# Autodesk Inventor assembly: Wind Tunnel Inlet Test Assembly (To Simulate)
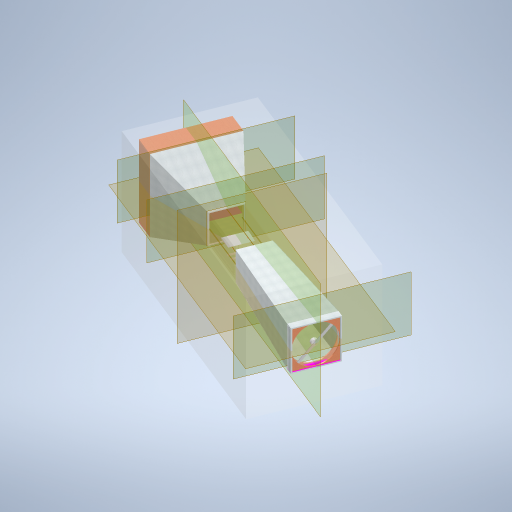
[picture p0: Inventor's stored thumbnail of the model, 512x512]
Saved by Autodesk Inventor 2023 (Build 270158000, 158)
## iProperties
Created: 2022-01-10
Part Number: Wind Tunnel Inlet Test Assembly (To Simulate)
Document SubType Name: Assembly
Designer: kamer
Author: kamer
## iProperties of the stored document MemberDocs/xAaaaqwbaAaaaaaaaAaaaavk0Cc
Created: 2022-01-10
Part Number: Wind Tunnel Inlet Test Assembly (To Simulate)
Document SubType Name: Assembly
Designer: kamer
Author: kamer
## Documents named in this file (21)
- X:\Storage\Documents\ME 306 Heat Transfer Project Files\CAD\Main With Subparts.iam
- X:\Storage\Documents\ME 306 Heat Transfer Project Files\CAD\Wind Tunnel Inlet Body Single Panel.ipt
- X:\Storage\Documents\ME 306 Heat Transfer Project Files\CAD\Wind Tunnel Output Body Single Panel.ipt
- X:\Storage\Documents\ME 306 Heat Transfer Project Files\CAD\Test Section Assembly.iam
- X:\Storage\Documents\ME 306 Heat Transfer Project Files\CAD\Fluid Simulation Boundary.ipt
- X:\Storage\Documents\ME 306 Heat Transfer Project Files\CAD\Wind Tunnel Settling Chamber.iam
- X:\Storage\Documents\ME 306 Heat Transfer Project Files\CAD\Wind Tunnel Exhaust Frame.iam
- X:\Storage\Documents\ME 306 Heat Transfer Project Files\CAD\Motor Mockup.ipt
- X:\Storage\Documents\ME 306 Heat Transfer Project Files\CAD\Wind Tunnel Fan Shroud Corner.ipt
- X:\Storage\Documents\ME 306 Heat Transfer Project Files\CAD\Motor Strap.ipt
- X:\Storage\Documents\ME 306 Heat Transfer Project Files\CAD\Wind Tunnel Exhaust Frame As-built.iam
- X:\Storage\Documents\ME 306 Heat Transfer Project Files\CAD\Wind Tunnel Inlet Body Single Panel Graphic Only.ipt
- X:\Storage\Documents\ME 306 Heat Transfer Project Files\CAD\Wind Tunnel Output Body Single Panel Graphic Only.ipt
- X:\Storage\Documents\ME 306 Heat Transfer Project Files\CAD\Wind Tunnel Settling Chamber As-Built.iam
- X:\Storage\Documents\ME 306 Heat Transfer Project Files\CAD\Inlet Support Leg Proto 1.ipt
- X:\Storage\Documents\ME 306 Heat Transfer Project Files\CAD\Outlet Support Leg Proto 1.ipt
- X:\Storage\Documents\ME 306 Heat Transfer Project Files\CAD\Computer Box Assembly Rev2.iam
- X:\Storage\Documents\ME 306 Heat Transfer Project Files\CAD\PowerBoardAssembly.iam
- X:\Storage\Documents\ME 306 Heat Transfer Project Files\CAD\Antitorque Outlet Support.ipt
- X:\Storage\Documents\ME 306 Heat Transfer Project Files\CAD\Antitorque span.ipt
- X:\Storage\Documents\ME 306 Heat Transfer Project Files\CAD\Antitorque leg-leg span.ipt
## Components (22 placed, 9 different names)
1. Wind Tunnel Inlet Body Single Panel:1 — Mate:1, Mate:3, Angle:1, Mate:24
2. Wind Tunnel Inlet Body Single Panel:2 — Mate:1, Mate:2, Angle:1, Mate:22, Mate:30, Mate:33
3. Wind Tunnel Inlet Body Single Panel:3 — Mate:2, Mate:4, Mate:14, Mate:23, Mate:32
4. Wind Tunnel Inlet Body Single Panel:4 — Mate:3, Mate:4, Mate:13, Mate:15, Mate:27
5. Wind Tunnel Output Body Single Panel:1 — Mate:16, Mate:17, Mate:22, Mate:35
6. Wind Tunnel Output Body Single Panel:2 — Mate:18, Mate:19, Mate:24, Mate:34
7. Wind Tunnel Output Body Single Panel:3 — Mate:25, Mate:26, Mate:27
8. Wind Tunnel Output Body Single Panel:4 — Mate:20, Mate:21, Mate:23
9. Test Section Assembly:1 [sub-assembly] — Mate:13, Mate:14, Mate:15, Mate:16, Mate:17, Mate:18, Mate:19, Mate:20, Mate:21, Mate:25, Mate:26, Mate:28, Mate:29, Angle:2
10. Fluid Simulation Boundary:1 — Mate:28, Mate:29
11. Wind Tunnel Settling Chamber:1 [sub-assembly] — Mate:31, Mate:32, Mate:33
12. Wind Tunnel Exhaust Frame:1 [sub-assembly] — Flush:3, Mate:34, Mate:35, Mate:36, Mate:37, Flush:4, Mate:38, Mate:39, Mate:40, Mate:41, Mate:42, Mate:43, Mate:47, Mate:48, Mate:50, Mate:51, Mate:52, Mate:53, Mate:56, Mate:57, Mate:58, Mate:59
13. Motor Mockup:1 — Mate:44, Mate:45, Mate:49
14. Wind Tunnel Fan Shroud Corner:1 — Mate:36, Mate:37, Flush:4, Flush:5, Mate:45
15. Wind Tunnel Fan Shroud Corner:2 — Mate:42, Mate:43, Flush:7, Mate:44
16. Wind Tunnel Fan Shroud Corner:3 — Mate:40, Mate:41, Flush:6, Flush:7
17. Wind Tunnel Fan Shroud Corner:4 — Mate:38, Mate:39, Flush:5, Flush:6
18. Motor Strap:1 — Mate:47, Mate:48, Mate:49, Mate:54, Mate:55
19. Wind Tunnel Fan Shroud Corner:5 — Mate:50, Mate:51, Mate:54, Flush:8
20. Wind Tunnel Fan Shroud Corner:6 — Mate:52, Mate:53, Mate:55, Flush:9
21. Wind Tunnel Fan Shroud Corner:7 — Mate:56, Mate:57, Flush:8
22. Wind Tunnel Fan Shroud Corner:8 — Mate:58, Mate:59, Flush:9
## Relationships (61: Mate 50, Flush 9, Angle 2)
- Mate:1: Wind Tunnel Inlet Body Single Panel:1 ↔ Wind Tunnel Inlet Body Single Panel:2
- Mate:2: Wind Tunnel Inlet Body Single Panel:2 ↔ Wind Tunnel Inlet Body Single Panel:3
- Mate:3: Wind Tunnel Inlet Body Single Panel:1 ↔ Wind Tunnel Inlet Body Single Panel:4
- Mate:4: Wind Tunnel Inlet Body Single Panel:3 ↔ Wind Tunnel Inlet Body Single Panel:4
- Angle:1 (90 deg): Wind Tunnel Inlet Body Single Panel:1 ↔ Wind Tunnel Inlet Body Single Panel:2
- Mate:13: Wind Tunnel Inlet Body Single Panel:4 ↔ Test Section Assembly:1
- Mate:14: Wind Tunnel Inlet Body Single Panel:3 ↔ Test Section Assembly:1
- Mate:15: Wind Tunnel Inlet Body Single Panel:4 ↔ Test Section Assembly:1
- Mate:16: Wind Tunnel Output Body Single Panel:1 ↔ Test Section Assembly:1
- Mate:17: Wind Tunnel Output Body Single Panel:1 ↔ Test Section Assembly:1
- Mate:18: Wind Tunnel Output Body Single Panel:2 ↔ Test Section Assembly:1
- Mate:19: Wind Tunnel Output Body Single Panel:2 ↔ Test Section Assembly:1
- Mate:20: Wind Tunnel Output Body Single Panel:4 ↔ Test Section Assembly:1
- Mate:21: Wind Tunnel Output Body Single Panel:4 ↔ Test Section Assembly:1
- Mate:22: Wind Tunnel Inlet Body Single Panel:2 ↔ Wind Tunnel Output Body Single Panel:1
- Mate:23: Wind Tunnel Inlet Body Single Panel:3 ↔ Wind Tunnel Output Body Single Panel:4
- Mate:24: Wind Tunnel Inlet Body Single Panel:1 ↔ Wind Tunnel Output Body Single Panel:2
- Mate:25: Wind Tunnel Output Body Single Panel:3 ↔ Test Section Assembly:1
- Mate:26: Wind Tunnel Output Body Single Panel:3 ↔ Test Section Assembly:1
- Mate:27: Wind Tunnel Inlet Body Single Panel:4 ↔ Wind Tunnel Output Body Single Panel:3
- Mate:28: Test Section Assembly:1 ↔ Fluid Simulation Boundary:1
- Mate:29: Test Section Assembly:1 ↔ Fluid Simulation Boundary:1
- Mate:30: Wind Tunnel Inlet Body Single Panel:2
- Angle:2 (90 deg): Test Section Assembly:1
- Flush:1 (617.22 mm)
- Mate:31: Wind Tunnel Settling Chamber:1
- Mate:32: Wind Tunnel Inlet Body Single Panel:3 ↔ Wind Tunnel Settling Chamber:1
- Mate:33: Wind Tunnel Inlet Body Single Panel:2 ↔ Wind Tunnel Settling Chamber:1
- Flush:2 (-1801.0886 mm)
- Flush:3: Wind Tunnel Exhaust Frame:1
- Mate:34: Wind Tunnel Output Body Single Panel:2 ↔ Wind Tunnel Exhaust Frame:1
- Mate:35: Wind Tunnel Output Body Single Panel:1 ↔ Wind Tunnel Exhaust Frame:1
- Mate:36: Wind Tunnel Exhaust Frame:1 ↔ Wind Tunnel Fan Shroud Corner:1
- Mate:37: Wind Tunnel Exhaust Frame:1 ↔ Wind Tunnel Fan Shroud Corner:1
- Flush:4 (63.5 mm): Wind Tunnel Exhaust Frame:1 ↔ Wind Tunnel Fan Shroud Corner:1
- Mate:38: Wind Tunnel Exhaust Frame:1 ↔ Wind Tunnel Fan Shroud Corner:4
- Mate:39: Wind Tunnel Exhaust Frame:1 ↔ Wind Tunnel Fan Shroud Corner:4
- Flush:5: Wind Tunnel Fan Shroud Corner:1 ↔ Wind Tunnel Fan Shroud Corner:4
- Mate:40: Wind Tunnel Exhaust Frame:1 ↔ Wind Tunnel Fan Shroud Corner:3
- Mate:41: Wind Tunnel Exhaust Frame:1 ↔ Wind Tunnel Fan Shroud Corner:3
- Flush:6: Wind Tunnel Fan Shroud Corner:3 ↔ Wind Tunnel Fan Shroud Corner:4
- Mate:42: Wind Tunnel Exhaust Frame:1 ↔ Wind Tunnel Fan Shroud Corner:2
- Mate:43: Wind Tunnel Exhaust Frame:1 ↔ Wind Tunnel Fan Shroud Corner:2
- Flush:7: Wind Tunnel Fan Shroud Corner:2 ↔ Wind Tunnel Fan Shroud Corner:3
- Mate:44: Motor Mockup:1 ↔ Wind Tunnel Fan Shroud Corner:2
- Mate:45: Motor Mockup:1 ↔ Wind Tunnel Fan Shroud Corner:1
- Mate:47: Wind Tunnel Exhaust Frame:1 ↔ Motor Strap:1
- Mate:48: Wind Tunnel Exhaust Frame:1 ↔ Motor Strap:1
- Mate:49: Motor Mockup:1 ↔ Motor Strap:1
- Mate:50: Wind Tunnel Exhaust Frame:1 ↔ Wind Tunnel Fan Shroud Corner:5
- Mate:51: Wind Tunnel Exhaust Frame:1 ↔ Wind Tunnel Fan Shroud Corner:5
- Mate:52: Wind Tunnel Exhaust Frame:1 ↔ Wind Tunnel Fan Shroud Corner:6
- Mate:53: Wind Tunnel Exhaust Frame:1 ↔ Wind Tunnel Fan Shroud Corner:6
- Mate:54: Motor Strap:1 ↔ Wind Tunnel Fan Shroud Corner:5
- Mate:55: Motor Strap:1 ↔ Wind Tunnel Fan Shroud Corner:6
- Mate:56: Wind Tunnel Exhaust Frame:1 ↔ Wind Tunnel Fan Shroud Corner:7
- Mate:57: Wind Tunnel Exhaust Frame:1 ↔ Wind Tunnel Fan Shroud Corner:7
- Flush:8: Wind Tunnel Fan Shroud Corner:5 ↔ Wind Tunnel Fan Shroud Corner:7
- Mate:58: Wind Tunnel Exhaust Frame:1 ↔ Wind Tunnel Fan Shroud Corner:8
- Mate:59: Wind Tunnel Exhaust Frame:1 ↔ Wind Tunnel Fan Shroud Corner:8
- Flush:9: Wind Tunnel Fan Shroud Corner:6 ↔ Wind Tunnel Fan Shroud Corner:8
